# Autodesk Inventor assembly: containerBulkheadAssy
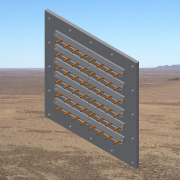
[picture p0: Inventor's stored thumbnail of the model, 180x180]
Saved by Autodesk Inventor 2014 SP1 (Build 180222100, 222)
## iProperties
Created: 2013-04-24
Part Number: containerBulkheadAssy
Document SubType Name: Assembly
Designer: Dave
Author: Dave
## Documents named in this file (4)
- C:\Users\Dave\Desktop\PAPER\2013deploy\containerBulkheadAssy.iam
- C:\Users\Dave\Desktop\PAPER\2013deploy\plate.ipt
- C:\Users\Dave\Desktop\PAPER\2013deploy\bar.ipt
- C:\Users\Dave\Desktop\PAPER\2013deploy\sma_female_bulkhead.ipt
## Components (55 placed, 3 different names)
1. plate:1 — Mate:5
2. bar:1
3. bar:2
4. bar:3
5. bar:4
6. bar:5
7. bar:6
8. sma_female_bulkhead:1 — Mate:5
9. sma_female_bulkhead:2
10. sma_female_bulkhead:3
11. sma_female_bulkhead:4
12. sma_female_bulkhead:5
13. sma_female_bulkhead:6
14. sma_female_bulkhead:7
15. sma_female_bulkhead:8
16. sma_female_bulkhead:9
17. sma_female_bulkhead:10
18. sma_female_bulkhead:11
19. sma_female_bulkhead:12
20. sma_female_bulkhead:13
21. sma_female_bulkhead:14
22. sma_female_bulkhead:15
23. sma_female_bulkhead:16
24. sma_female_bulkhead:17
25. sma_female_bulkhead:18
26. sma_female_bulkhead:19
27. sma_female_bulkhead:20
28. sma_female_bulkhead:21
29. sma_female_bulkhead:22
30. sma_female_bulkhead:23
31. sma_female_bulkhead:24
32. sma_female_bulkhead:25
33. sma_female_bulkhead:26
34. sma_female_bulkhead:27
35. sma_female_bulkhead:28
36. sma_female_bulkhead:29
37. sma_female_bulkhead:30
38. sma_female_bulkhead:31
39. sma_female_bulkhead:32
40. sma_female_bulkhead:33
41. sma_female_bulkhead:34
42. sma_female_bulkhead:35
43. sma_female_bulkhead:36
44. sma_female_bulkhead:37
45. sma_female_bulkhead:38
46. sma_female_bulkhead:39
47. sma_female_bulkhead:40
48. sma_female_bulkhead:41
49. sma_female_bulkhead:42
50. sma_female_bulkhead:43
51. sma_female_bulkhead:44
52. sma_female_bulkhead:45
53. sma_female_bulkhead:46
54. sma_female_bulkhead:47
55. sma_female_bulkhead:48
## Component patterns: (48 elements, first: sma_female_bulkhead:1)
## Relationships (1: Mate 1)
- Mate:5: plate:1 ↔ sma_female_bulkhead:1
